# Autodesk Inventor assembly: 足ユニット_MIR
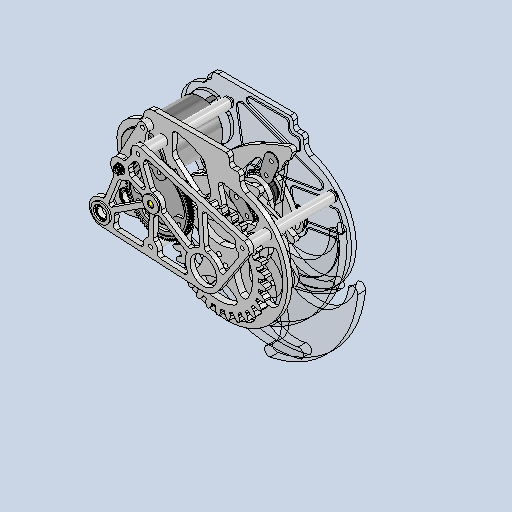
[picture p0: Inventor's stored thumbnail of the model, 512x512]
Saved by Autodesk Inventor 2023 (Build 270158000, 158)
## iProperties
Created: 2022-01-10
Part Number: 足ユニット_MIR
Document SubType Name: Assembly
Designer: acps
Author: acps
## Documents named in this file (20)
- C:\Users\acps\Documents\srdc\srdc_ksh\脚\足ユニット_MIR.iam
- C:\Users\acps\Documents\srdc\srdc_ksh\スペーサ\l40.ipt
- C:\Users\acps\Documents\srdc\srdc_ksh\カム\カム4.ipt
- C:\Users\acps\Documents\srdc\srdc_ksh\オイレス\w5f15-17n.ipt
- C:\Users\acps\Documents\srdc\srdc_ksh\モータ\M-RS-380_MIR.ipt
- C:\Users\acps\Documents\srdc\srdc_ksh\ベアリング\φ6φ12ベアリングa.ipt
- C:\Users\acps\Documents\srdc\srdc_ksh\脚\モータマウント_MIR.ipt
- C:\Users\acps\Documents\srdc\srdc_ksh\脚\ギア\ぴにょん.ipt
- C:\Users\acps\Documents\srdc\srdc_ksh\ベアリング\M-φ4φ8a.ipt
- C:\Users\acps\Documents\srdc\srdc_ksh\脚\ギア\初段_多段ギア.iam
- C:\Users\acps\Documents\srdc\srdc_ksh\ピン\φ4ピン　L20.ipt
- C:\Users\acps\Documents\srdc\srdc_ksh\ベアリング\φ4φ8ベアリングa.ipt
- C:\Users\acps\Documents\srdc\srdc_ksh\脚\ギア\最終段m2z28t4.ipt
- C:\Users\acps\Documents\srdc\srdc_ksh\脚\クランク_MIR.iam
- C:\Users\acps\Documents\srdc\srdc_ksh\脚\揺動節+ヘッケン_MIR.iam
- C:\Users\acps\Documents\srdc\srdc_ksh\スペーサ\l14.ipt
- C:\Users\acps\Documents\srdc\srdc_ksh\脚\足外フレーム_MIR.ipt
- C:\Users\acps\Documents\srdc\srdc_ksh\脚\ギア抑え_MIR.ipt
- C:\Users\acps\Documents\srdc\srdc_ksh\脚\足内フレーム_MIR.ipt
- C:\Users\acps\Documents\srdc\srdc_ksh\ベアリング\φ6φ10ベアリングa.ipt
## Components (27 placed, 19 different names)
1. l40:1 — Insert:68, Mate:72
2. l40:2 — Insert:67
3. l40:3 — Mate:51, Mate:53, Mate:55, Mate:49, Insert:65, Mate:64
4. カム4:1 — Insert:9, Insert:75, Mate:70, Mate:69, Mate:68, Insert:51
5. w5f15-17n:1 — Insert:9
6. M-RS-380_MIR:1 — Mate:71, Mate:61, Insert:31, Insert:32, Mate:38, Mate:62
7. φ6φ12ベアリングa:1 — Insert:86
8. モータマウント_MIR:1 — Mate:71, Mate:61, Insert:31, Mate:76, Insert:83
9. ぴにょん:1 — Insert:32, Mate:38
10. M-φ4φ8a:1 — Mate:41, Insert:81, Mate:42, Insert:80
11. 初段_多段ギア:1 [sub-assembly] — Mate:62, Mate:41
12. φ4ピン　L20:1 — Insert:81, Mate:42
13. φ4φ8ベアリングa:1
14. 最終段m2z28t4:1 — Insert:75, Mate:70, Mate:69
15. クランク_MIR:1 [sub-assembly] — Mate:68, Insert:51, Insert:54, Mate:52, Insert:55, Mate:54, Insert:56, Mate:56, Insert:52, Mate:50
16. 揺動節+ヘッケン_MIR:1 [sub-assembly] — Insert:54, Mate:52, Mate:51
17. 揺動節+ヘッケン_MIR:2 [sub-assembly] — Insert:55, Mate:54, Mate:53
18. 揺動節+ヘッケン_MIR:3 [sub-assembly] — Insert:56, Mate:56, Mate:55
19. 揺動節+ヘッケン_MIR:4 [sub-assembly] — Insert:52, Mate:50, Mate:49
20. l14:1
21. l14:2 — Insert:79, Insert:82
22. l14:3
23. 足外フレーム_MIR:1 — Insert:86, Insert:68, Insert:67, Insert:65, Mate:64, Mate:75, Mate:74
24. ギア抑え_MIR:1 — Insert:80, Mate:72, Insert:79, Insert:84
25. 足内フレーム_MIR:1 — Mate:76, Insert:83, Insert:82, Mate:75, Mate:74, Insert:85
26. φ6φ10ベアリングa:1 — Insert:84
27. φ6φ10ベアリングa:2 — Insert:85
## Relationships (42: Mate 22, Insert 20)
- Insert:9: カム4:1 ↔ w5f15-17n:1
- Mate:71: M-RS-380_MIR:1 ↔ モータマウント_MIR:1
- Mate:61: M-RS-380_MIR:1 ↔ モータマウント_MIR:1
- Insert:31: M-RS-380_MIR:1 ↔ モータマウント_MIR:1
- Insert:32: M-RS-380_MIR:1 ↔ ぴにょん:1
- Mate:38: M-RS-380_MIR:1 ↔ ぴにょん:1
- Mate:62 (0.3 mm): M-RS-380_MIR:1 ↔ 初段_多段ギア:1
- Mate:41: M-φ4φ8a:1 ↔ 初段_多段ギア:1
- Insert:81 (0.5 mm): M-φ4φ8a:1 ↔ φ4ピン　L20:1
- Mate:42: M-φ4φ8a:1 ↔ φ4ピン　L20:1
- Insert:75: カム4:1 ↔ 最終段m2z28t4:1
- Mate:70: カム4:1 ↔ 最終段m2z28t4:1
- Mate:69: カム4:1 ↔ 最終段m2z28t4:1
- Mate:68: カム4:1 ↔ クランク_MIR:1
- Insert:51: カム4:1 ↔ クランク_MIR:1
- Insert:54 (0.25 mm): クランク_MIR:1 ↔ 揺動節+ヘッケン_MIR:1
- Mate:52: クランク_MIR:1 ↔ 揺動節+ヘッケン_MIR:1
- Mate:51: l40:3 ↔ 揺動節+ヘッケン_MIR:1
- Insert:55 (0.25 mm): クランク_MIR:1 ↔ 揺動節+ヘッケン_MIR:2
- Mate:54: クランク_MIR:1 ↔ 揺動節+ヘッケン_MIR:2
- Mate:53: l40:3 ↔ 揺動節+ヘッケン_MIR:2
- Insert:56 (0.25 mm): クランク_MIR:1 ↔ 揺動節+ヘッケン_MIR:3
- Mate:56: クランク_MIR:1 ↔ 揺動節+ヘッケン_MIR:3
- Mate:55: l40:3 ↔ 揺動節+ヘッケン_MIR:3
- Insert:52 (0.25 mm): クランク_MIR:1 ↔ 揺動節+ヘッケン_MIR:4
- Mate:50: クランク_MIR:1 ↔ 揺動節+ヘッケン_MIR:4
- Mate:49: l40:3 ↔ 揺動節+ヘッケン_MIR:4
- Insert:86: φ6φ12ベアリングa:1 ↔ 足外フレーム_MIR:1
- Insert:68: l40:1 ↔ 足外フレーム_MIR:1
- Insert:67: l40:2 ↔ 足外フレーム_MIR:1
- Insert:65: l40:3 ↔ 足外フレーム_MIR:1
- Mate:64: l40:3 ↔ 足外フレーム_MIR:1
- Insert:80: M-φ4φ8a:1 ↔ ギア抑え_MIR:1
- Mate:72: l40:1 ↔ ギア抑え_MIR:1
- Insert:79: l14:2 ↔ ギア抑え_MIR:1
- Mate:76: モータマウント_MIR:1 ↔ 足内フレーム_MIR:1
- Insert:83: モータマウント_MIR:1 ↔ 足内フレーム_MIR:1
- Insert:82: l14:2 ↔ 足内フレーム_MIR:1
- Mate:75: 足外フレーム_MIR:1 ↔ 足内フレーム_MIR:1
- Mate:74: 足外フレーム_MIR:1 ↔ 足内フレーム_MIR:1
- Insert:84: ギア抑え_MIR:1 ↔ φ6φ10ベアリングa:1
- Insert:85: 足内フレーム_MIR:1 ↔ φ6φ10ベアリングa:2
